# Autodesk Inventor assembly: PaddleCollection2.1.ipt
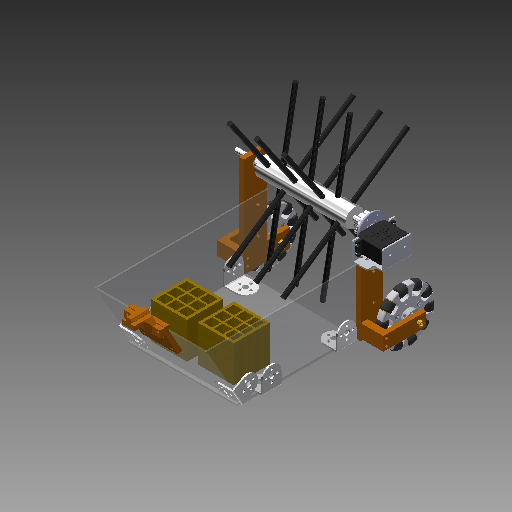
[picture p0: Inventor's stored thumbnail of the model, 512x512]
Saved by Autodesk Inventor 2019 (Build 230136000, 136)
## iProperties
Created: 2018-10-20
Part Number: PaddleCollection2.1.ipt
Document SubType Name: Assembly
Designer: User
Mass: 862.445 g
Surface Area: 4404.87 cm^2
Volume: 627.029 cm^3
Density: 1.37545 g/cm^3
Author: User
## Documents named in this file (24)
- C:\Robotics\CAD\2018-19_CAD\Collection\PaddleCollection2.1.ipt.iam
- C:\Robotics\CAD\2018-19_CAD\Collection\PaddleCollection2.1AxleSupport.ipt
- C:\Robotics\CAD\2018-19_CAD\Collection\PaddleCollection2.1Casing.ipt
- C:\Robotics\CAD\2018-19_CAD\Collection\PaddleCollectionFloor.ipt
- C:\Robotics\CAD\COTSParts\Tetrix\Tetrix Wheel 3 in omni.ipt
- C:\Robotics\CAD\COTSParts\Tetrix\Bronze bushing.ipt
- C:\Robotics\CAD\COTSParts\Tetrix\Tetrix shaft collar.ipt
- C:\Robotics\CAD\COTSParts\Tetrix\Tetrix Hub - axle.ipt
- C:\Robotics\CAD\COTSParts\Rev\REV-41-1097SmartServo.ipt
- C:\Robotics\CAD\COTSParts\Tetrix\39060_txm-standard servo bracket.ipt
- C:\Robotics\CAD\COTSParts\Tetrix\Tetrix bracket - angle.ipt
- C:\Robotics\CAD\2018-19_CAD\Collection\PaddleCollection2.1ServoSupport.ipt
- C:\Robotics\CAD\COTSParts\Bearings - AndyMark\Bearing 250 ID 500 OD flanged.ipt
- C:\Robotics\CAD\COTSParts\Actobotics\Collar.ipt
- C:\Robotics\CAD\COTSParts\Rev\REV-41-1363ServoHorn.ipt
- C:\Robotics\CAD\COTSParts\Actobotics\545 parts\545456PatternAdapter.77in.625in.ipt
- C:\Robotics\CAD\COTSParts\Actobotics\545 parts\545548SetScrewHub.77inPattern.ipt
- C:\Robotics\CAD\2018-19_CAD\Collection\SweeperAxle.ipt
- C:\Robotics\CAD\2018-19_CAD\Collection\SweeperSpoke.ipt
- C:\Robotics\CAD\2018-19_CAD\Collection\PaddleCollection2.1Backing.ipt
- C:\Robotics\CAD\2018-19_CAD\Field Pieces\Gold.ipt
- C:\Robotics\CAD\2018-19_CAD\Collection\PaddleCollection2.1WheelBracket.ipt
- C:\Robotics\CAD\2018-19_CAD\Collection\PaddleCollection2.1AngleBracket.ipt
- C:\Robotics\CAD\2018-19_CAD\Collection\PaddleCollection2.1SlidingConnector.ipt
## Components (46 placed, 23 different names)
1. PaddleCollection2.1AxleSupport:1 — Insert:1, Insert:42, Insert:43, Insert:46, Insert:47, Insert:51
2. PaddleCollection2.1Casing:1 — Angle:5, Insert:26, Insert:27, Insert:28, Insert:29, Insert:30, Insert:42, Insert:43
3. PaddleCollection2.1Casing:2 — Insert:21, Angle:3, Insert:22, Insert:23, Insert:24, Insert:25, Angle:4, Insert:44, Insert:45, Mate:49
4. PaddleCollectionFloor:1 — Mate:44, Mate:45, Insert:31, Insert:32, Insert:33, Insert:34, Insert:35, Insert:36, Insert:37
5. Tetrix Wheel 3 in omni:1 — Insert:3, Insert:4
6. Bronze bushing:1 — Insert:1, Insert:2
7. Bronze bushing:2 — Insert:5
8. Tetrix shaft collar:1 — Insert:2, Insert:3
9. Tetrix Hub - axle:1 — Insert:4, Insert:5
10. REV-41-1097SmartServo:1 — Insert:6, Angle:1, Insert:17
11. 39060_txm-standard servo bracket:1 — Insert:6, Angle:1, Insert:7, Insert:8
12. Tetrix bracket - angle:1 — Insert:7, Insert:8, Insert:9, Angle:2
13. PaddleCollection2.1ServoSupport:1 — Insert:9, Angle:2, Insert:10, Insert:44, Insert:45, Insert:48, Insert:49
14. Bronze bushing:3 — Insert:14
15. Tetrix Wheel 3 in omni:2 — Insert:12, Insert:13
16. Tetrix shaft collar:2 — Insert:11, Insert:12
17. Tetrix Hub - axle:2 — Insert:13, Insert:14
18. Bronze bushing:4 — Insert:10, Insert:11
19. Collar:1 — Mate:46, Mate:50
20. Tetrix bracket - angle:2 — Insert:23, Insert:24, Insert:37
21. Tetrix bracket - angle:3 — Insert:29, Insert:30, Insert:33, Insert:34
22. REV-41-1363ServoHorn:1 — Insert:17, Insert:18
23. 545456PatternAdapter.77in.625in:1 — Insert:18, Insert:19
24. 545548SetScrewHub.77inPattern:1 — Insert:19, Insert:20
25. SweeperAxle:1 — Mate:15, Mate:16, Mate:17, Mate:18, Mate:19, Mate:20, Mate:21, Mate:22, Mate:23, Mate:24, Mate:25, Mate:26, Mate:27, Mate:28, Mate:29, Mate:30, Mate:31, Mate:32, Mate:33, Insert:20, Mate:46, Mate:50
26. SweeperSpoke:1 — Mate:19, Mate:32
27. SweeperSpoke:2 — Mate:18, Mate:31
28. SweeperSpoke:3 — Mate:17, Mate:25
29. SweeperSpoke:4 — Mate:21, Mate:27, Mate:28
30. SweeperSpoke:5 — Mate:22, Mate:26
31. SweeperSpoke:6 — Mate:23, Mate:33
32. SweeperSpoke:7 — Mate:24, Mate:30
33. SweeperSpoke:8 — Mate:20, Mate:29
34. SweeperSpoke:9 — Mate:15, Mate:16
35. PaddleCollection2.1Backing:1 — Insert:38, Insert:39, Insert:40, Insert:41, Mate:47, Mate:48
36. Tetrix bracket - angle:4 — Insert:21, Angle:3, Insert:22, Insert:35, Insert:36
37. Tetrix bracket - angle:5 — Insert:25, Angle:4, Insert:40, Insert:41
38. Tetrix bracket - angle:6 — Angle:5, Insert:26, Insert:38, Insert:39
39. Tetrix bracket - angle:7 — Insert:27, Insert:28, Insert:31, Insert:32
40. Gold:1 — Mate:44
41. Gold:2 — Mate:45
42. PaddleCollection2.1WheelBracket:1 — Insert:46, Insert:47
43. PaddleCollection2.1WheelBracket:2 — Insert:48, Insert:49
44. PaddleCollection2.1AngleBracket:1 — Mate:47, Mate:48, Mate:49, Insert:50, Angle:6
45. PaddleCollection2.1SlidingConnector:1 — Insert:50, Angle:6
46. Bearing 250 ID 500 OD flanged:2 — Insert:51
## Relationships (81: Insert 49, Mate 26, Angle 6)
- Insert:1: PaddleCollection2.1AxleSupport:1 ↔ Bronze bushing:1
- Insert:2: Bronze bushing:1 ↔ Tetrix shaft collar:1
- Insert:3: Tetrix Wheel 3 in omni:1 ↔ Tetrix shaft collar:1
- Insert:4: Tetrix Wheel 3 in omni:1 ↔ Tetrix Hub - axle:1
- Insert:5: Bronze bushing:2 ↔ Tetrix Hub - axle:1
- Insert:6: REV-41-1097SmartServo:1 ↔ 39060_txm-standard servo bracket:1
- Angle:1 (0 deg): REV-41-1097SmartServo:1 ↔ 39060_txm-standard servo bracket:1
- Insert:7: 39060_txm-standard servo bracket:1 ↔ Tetrix bracket - angle:1
- Insert:8: 39060_txm-standard servo bracket:1 ↔ Tetrix bracket - angle:1
- Insert:9: Tetrix bracket - angle:1 ↔ PaddleCollection2.1ServoSupport:1
- Angle:2 (0 deg): Tetrix bracket - angle:1 ↔ PaddleCollection2.1ServoSupport:1
- Insert:10: PaddleCollection2.1ServoSupport:1 ↔ Bronze bushing:4
- Insert:11: Tetrix shaft collar:2 ↔ Bronze bushing:4
- Insert:12: Tetrix Wheel 3 in omni:2 ↔ Tetrix shaft collar:2
- Insert:13: Tetrix Wheel 3 in omni:2 ↔ Tetrix Hub - axle:2
- Insert:14: Bronze bushing:3 ↔ Tetrix Hub - axle:2
- Insert:17: REV-41-1097SmartServo:1 ↔ REV-41-1363ServoHorn:1
- Insert:18: REV-41-1363ServoHorn:1 ↔ 545456PatternAdapter.77in.625in:1
- Insert:19: 545456PatternAdapter.77in.625in:1 ↔ 545548SetScrewHub.77inPattern:1
- Mate:15: SweeperAxle:1 ↔ SweeperSpoke:9
- Mate:16 (-106.3625 mm): SweeperAxle:1 ↔ SweeperSpoke:9
- Mate:17: SweeperAxle:1 ↔ SweeperSpoke:3
- Mate:18: SweeperAxle:1 ↔ SweeperSpoke:2
- Mate:19: SweeperAxle:1 ↔ SweeperSpoke:1
- Mate:20: SweeperAxle:1 ↔ SweeperSpoke:8
- Mate:21: SweeperAxle:1 ↔ SweeperSpoke:4
- Mate:22: SweeperAxle:1 ↔ SweeperSpoke:5
- Mate:23: SweeperAxle:1 ↔ SweeperSpoke:6
- Mate:24: SweeperAxle:1 ↔ SweeperSpoke:7
- Mate:25 (-106.3625 mm): SweeperAxle:1 ↔ SweeperSpoke:3
- Mate:26 (-106.3625 mm): SweeperAxle:1 ↔ SweeperSpoke:5
- Mate:27 (-106.3625 mm): SweeperAxle:1 ↔ SweeperSpoke:4
- Mate:28 (-106.3625 mm): SweeperAxle:1 ↔ SweeperSpoke:4
- Mate:29 (-106.3625 mm): SweeperAxle:1 ↔ SweeperSpoke:8
- Mate:30 (-106.3625 mm): SweeperAxle:1 ↔ SweeperSpoke:7
- Mate:31 (-106.3625 mm): SweeperAxle:1 ↔ SweeperSpoke:2
- Mate:32 (-106.3625 mm): SweeperAxle:1 ↔ SweeperSpoke:1
- Mate:33 (-106.3625 mm): SweeperAxle:1 ↔ SweeperSpoke:6
- Insert:20 (6.35 mm): 545548SetScrewHub.77inPattern:1 ↔ SweeperAxle:1
- Mate:44: PaddleCollectionFloor:1 ↔ Gold:1
- Mate:45: PaddleCollectionFloor:1 ↔ Gold:2
- Insert:21: PaddleCollection2.1Casing:2 ↔ Tetrix bracket - angle:4
- Angle:3 (0 deg): PaddleCollection2.1Casing:2 ↔ Tetrix bracket - angle:4
- Insert:22: PaddleCollection2.1Casing:2 ↔ Tetrix bracket - angle:4
- Insert:23: PaddleCollection2.1Casing:2 ↔ Tetrix bracket - angle:2
- Insert:24: PaddleCollection2.1Casing:2 ↔ Tetrix bracket - angle:2
- Insert:25: PaddleCollection2.1Casing:2 ↔ Tetrix bracket - angle:5
- Angle:4 (0 deg): PaddleCollection2.1Casing:2 ↔ Tetrix bracket - angle:5
- Angle:5 (0 deg): PaddleCollection2.1Casing:1 ↔ Tetrix bracket - angle:6
- Insert:26: PaddleCollection2.1Casing:1 ↔ Tetrix bracket - angle:6
- Insert:27: PaddleCollection2.1Casing:1 ↔ Tetrix bracket - angle:7
- Insert:28: PaddleCollection2.1Casing:1 ↔ Tetrix bracket - angle:7
- Insert:29: PaddleCollection2.1Casing:1 ↔ Tetrix bracket - angle:3
- Insert:30: PaddleCollection2.1Casing:1 ↔ Tetrix bracket - angle:3
- Insert:31: PaddleCollectionFloor:1 ↔ Tetrix bracket - angle:7
- Insert:32: PaddleCollectionFloor:1 ↔ Tetrix bracket - angle:7
- Insert:33: PaddleCollectionFloor:1 ↔ Tetrix bracket - angle:3
- Insert:34: PaddleCollectionFloor:1 ↔ Tetrix bracket - angle:3
- Insert:35: PaddleCollectionFloor:1 ↔ Tetrix bracket - angle:4
- Insert:36: PaddleCollectionFloor:1 ↔ Tetrix bracket - angle:4
- Insert:37: PaddleCollectionFloor:1 ↔ Tetrix bracket - angle:2
- Insert:38: PaddleCollection2.1Backing:1 ↔ Tetrix bracket - angle:6
- Insert:39: PaddleCollection2.1Backing:1 ↔ Tetrix bracket - angle:6
- Insert:40: PaddleCollection2.1Backing:1 ↔ Tetrix bracket - angle:5
- Insert:41: PaddleCollection2.1Backing:1 ↔ Tetrix bracket - angle:5
- Mate:46: Collar:1 ↔ SweeperAxle:1
- Insert:42: PaddleCollection2.1AxleSupport:1 ↔ PaddleCollection2.1Casing:1
- Insert:43: PaddleCollection2.1AxleSupport:1 ↔ PaddleCollection2.1Casing:1
- Insert:44: PaddleCollection2.1Casing:2 ↔ PaddleCollection2.1ServoSupport:1
- Insert:45: PaddleCollection2.1Casing:2 ↔ PaddleCollection2.1ServoSupport:1
- Insert:46: PaddleCollection2.1AxleSupport:1 ↔ PaddleCollection2.1WheelBracket:1
- Insert:47: PaddleCollection2.1AxleSupport:1 ↔ PaddleCollection2.1WheelBracket:1
- Insert:48: PaddleCollection2.1ServoSupport:1 ↔ PaddleCollection2.1WheelBracket:2
- Insert:49: PaddleCollection2.1ServoSupport:1 ↔ PaddleCollection2.1WheelBracket:2
- Mate:47: PaddleCollection2.1Backing:1 ↔ PaddleCollection2.1AngleBracket:1
- Mate:48: PaddleCollection2.1Backing:1 ↔ PaddleCollection2.1AngleBracket:1
- Mate:49 (50.8 mm): PaddleCollection2.1Casing:2 ↔ PaddleCollection2.1AngleBracket:1
- Insert:50: PaddleCollection2.1AngleBracket:1 ↔ PaddleCollection2.1SlidingConnector:1
- Angle:6 (180 deg): PaddleCollection2.1AngleBracket:1 ↔ PaddleCollection2.1SlidingConnector:1
- Insert:51: PaddleCollection2.1AxleSupport:1 ↔ Bearing 250 ID 500 OD flanged:2
- Mate:50: Collar:1 ↔ SweeperAxle:1
